# Autodesk Inventor assembly: 20-100-ALUPROFIL-CASE
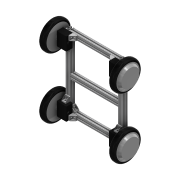
[picture p0: Inventor's stored thumbnail of the model, 180x180]
Saved by Autodesk Inventor 2018.1 (Build 221171000, 171)
## iProperties
Created: 2017-08-13
Part Number: 20-100-ALUPROFIL-CASE
Document SubType Name: Assembly
Designer: feesmrt
Author: feesmrt
## Documents named in this file (6)
- C:\Users\feesmrt\Documents\NRBDL\Inventor-NRBDL\20-CASE\20-100-ALUPROFIL-CASE.iam
- C:\Users\feesmrt\Documents\NRBDL\Inventor-NRBDL\20-CASE\20-006-30x30x450mm.ipt
- C:\Users\feesmrt\Documents\NRBDL\Inventor-NRBDL\20-CASE\20-007-30x30x290mm.ipt
- C:\Users\feesmrt\Documents\NRBDL\Inventor-NRBDL\20-CASE\WINKEL_30X30.ipt
- C:\Users\feesmrt\Documents\NRBDL\Inventor-NRBDL\10-SUSP\10-SUSP-PROFILE.iam
- C:\Users\feesmrt\Documents\NRBDL\Inventor-NRBDL\10-SUSP\10-SUSP-PROFILE-02.iam
## Components (13 placed, 5 different names)
1. 20-006-30x30x450mm:1 — Passend:1, Fluchtend:1, Fluchtend:2, Fluchtend:5, Passend:3, Fluchtend:6, Passend:5, Fluchtend:7, Passend:6, Fluchtend:8, Passend:12, Fluchtend:11, Passend:15, Fluchtend:18
2. 20-007-30x30x290mm:1 — Passend:1, Fluchtend:1, Fluchtend:2, Passend:2, Fluchtend:3, Fluchtend:4, Passend:4, Passend:10, Fluchtend:10, Fluchtend:12, Fluchtend:15, Passend:16
3. 20-006-30x30x450mm:2 — Passend:2, Fluchtend:3, Fluchtend:4, Passend:9, Passend:11, Passend:13, Fluchtend:13, Fluchtend:14, Passend:14, Fluchtend:16, Fluchtend:21, Passend:17
4. 20-007-30x30x290mm:2 — Fluchtend:5, Passend:3, Fluchtend:6, Passend:7, Passend:8, Fluchtend:9, Fluchtend:17
5. WINKEL_30X30:1 — Passend:4, Passend:5, Fluchtend:7
6. WINKEL_30X30:2 — Passend:6, Passend:7, Fluchtend:8
7. WINKEL_30X30:3 — Passend:8, Passend:9, Fluchtend:9
8. WINKEL_30X30:4 — Passend:10, Passend:11, Fluchtend:10
9. 10-SUSP-PROFILE:1 [sub-assembly] — Passend:12, Fluchtend:11, Fluchtend:12
10. 10-SUSP-PROFILE:2 [sub-assembly] — Passend:13, Fluchtend:13, Fluchtend:14
11. 10-SUSP-PROFILE-02:1 [sub-assembly] — Passend:14, Fluchtend:15, Fluchtend:16
12. 10-SUSP-PROFILE-02:2 [sub-assembly] — Passend:15, Fluchtend:17, Fluchtend:18
13. 20-007-30x30x290mm:3 — Fluchtend:21, Passend:16, Passend:17
## Relationships (36: Flush 19, Mate 17)
- Passend:1 [Mate]: 20-006-30x30x450mm:1 ↔ 20-007-30x30x290mm:1
- Fluchtend:1 [Flush]: 20-006-30x30x450mm:1 ↔ 20-007-30x30x290mm:1
- Fluchtend:2 [Flush]: 20-006-30x30x450mm:1 ↔ 20-007-30x30x290mm:1
- Passend:2 [Mate]: 20-007-30x30x290mm:1 ↔ 20-006-30x30x450mm:2
- Fluchtend:3 [Flush]: 20-007-30x30x290mm:1 ↔ 20-006-30x30x450mm:2
- Fluchtend:4 [Flush]: 20-007-30x30x290mm:1 ↔ 20-006-30x30x450mm:2
- Fluchtend:5 [Flush]: 20-006-30x30x450mm:1 ↔ 20-007-30x30x290mm:2
- Passend:3 [Mate]: 20-006-30x30x450mm:1 ↔ 20-007-30x30x290mm:2
- Fluchtend:6 [Flush]: 20-006-30x30x450mm:1 ↔ 20-007-30x30x290mm:2
- Passend:4 [Mate]: 20-007-30x30x290mm:1 ↔ WINKEL_30X30:1
- Passend:5 [Mate]: 20-006-30x30x450mm:1 ↔ WINKEL_30X30:1
- Fluchtend:7 [Flush]: 20-006-30x30x450mm:1 ↔ WINKEL_30X30:1
- Passend:6 [Mate]: 20-006-30x30x450mm:1 ↔ WINKEL_30X30:2
- Passend:7 [Mate]: 20-007-30x30x290mm:2 ↔ WINKEL_30X30:2
- Fluchtend:8 [Flush]: 20-006-30x30x450mm:1 ↔ WINKEL_30X30:2
- Passend:8 [Mate]: 20-007-30x30x290mm:2 ↔ WINKEL_30X30:3
- Passend:9 [Mate]: 20-006-30x30x450mm:2 ↔ WINKEL_30X30:3
- Fluchtend:9 [Flush]: 20-007-30x30x290mm:2 ↔ WINKEL_30X30:3
- Passend:10 [Mate]: 20-007-30x30x290mm:1 ↔ WINKEL_30X30:4
- Passend:11 [Mate]: 20-006-30x30x450mm:2 ↔ WINKEL_30X30:4
- Fluchtend:10 [Flush]: 20-007-30x30x290mm:1 ↔ WINKEL_30X30:4
- Passend:12 [Mate]: 20-006-30x30x450mm:1 ↔ 10-SUSP-PROFILE:1
- Fluchtend:11 [Flush]: 20-006-30x30x450mm:1 ↔ 10-SUSP-PROFILE:1
- Fluchtend:12 [Flush]: 20-007-30x30x290mm:1 ↔ 10-SUSP-PROFILE:1
- Passend:13 [Mate]: 20-006-30x30x450mm:2 ↔ 10-SUSP-PROFILE:2
- Fluchtend:13 [Flush]: 20-006-30x30x450mm:2 ↔ 10-SUSP-PROFILE:2
- Fluchtend:14 [Flush]: 20-006-30x30x450mm:2 ↔ 10-SUSP-PROFILE:2
- Passend:14 [Mate]: 20-006-30x30x450mm:2 ↔ 10-SUSP-PROFILE-02:1
- Fluchtend:15 [Flush]: 20-007-30x30x290mm:1 ↔ 10-SUSP-PROFILE-02:1
- Fluchtend:16 [Flush]: 20-006-30x30x450mm:2 ↔ 10-SUSP-PROFILE-02:1
- Passend:15 [Mate]: 20-006-30x30x450mm:1 ↔ 10-SUSP-PROFILE-02:2
- Fluchtend:17 [Flush]: 20-007-30x30x290mm:2 ↔ 10-SUSP-PROFILE-02:2
- Fluchtend:18 [Flush]: 20-006-30x30x450mm:1 ↔ 10-SUSP-PROFILE-02:2
- Fluchtend:21 [Flush]: 20-006-30x30x450mm:2 ↔ 20-007-30x30x290mm:3
- Passend:16 [Mate] (195 mm): 20-007-30x30x290mm:1 ↔ 20-007-30x30x290mm:3
- Passend:17 [Mate]: 20-006-30x30x450mm:2 ↔ 20-007-30x30x290mm:3
